# Autodesk Inventor assembly: DishBoard
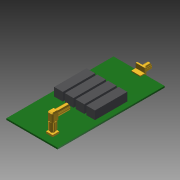
[picture p0: Inventor's stored thumbnail of the model, 180x180]
Saved by Autodesk Inventor 2014 (Build 180170000, 170)
## iProperties
Created: 2015-01-07
Part Number: DishBoard
Document SubType Name: Assembly
Designer: Owner
Author: Owner
## Documents named in this file (6)
- C:\Users\Owner\Documents\APC\FrontEnd\IAM\Dish\DishBoard.iam
- C:\Users\Owner\Documents\APC\FrontEnd\IAM\Dish\Dish_Board.ipt
- C:\Users\Owner\Documents\APC\FrontEnd\IAM\Common\SMA_Edge.ipt
- C:\Users\Owner\Documents\APC\FrontEnd\IAM\Common\SMA_Up.ipt
- C:\Users\Owner\Documents\APC\FrontEnd\IAM\Common\SMA_RightAngle.ipt
- C:\Users\Owner\Documents\APC\FrontEnd\IAM\Common\BPF.ipt
## Components (8 placed, 5 different names)
1. Dish_Board:1 — Mate:3, Mate:4, Flush:3, Mate:12, Mate:13, Mate:14, Mate:15, Mate:16, Flush:4, Flush:5, Flush:6, Flush:7, Flush:8, Flush:9, Flush:10, Flush:11
2. SMA_Edge:4 — Mate:3, Mate:4, Flush:3
3. SMA_Up:1 — Mate:10, Mate:11, Mate:12
4. SMA_RightAngle:1 — Mate:10, Mate:11
5. BPF:1 — Mate:13, Flush:7, Flush:11
6. BPF:2 — Mate:14, Flush:5, Flush:8
7. BPF:3 — Mate:15, Flush:4, Flush:10
8. BPF:4 — Mate:16, Flush:6, Flush:9
## Relationships (18: Mate 9, Flush 9)
- Mate:3: Dish_Board:1 ↔ SMA_Edge:4
- Mate:4: Dish_Board:1 ↔ SMA_Edge:4
- Flush:3 (-21.336 mm): Dish_Board:1 ↔ SMA_Edge:4
- Mate:10 (2 mm): SMA_Up:1 ↔ SMA_RightAngle:1
- Mate:11: SMA_Up:1 ↔ SMA_RightAngle:1
- Mate:12: Dish_Board:1 ↔ SMA_Up:1
- Mate:13: Dish_Board:1 ↔ BPF:1
- Mate:14: Dish_Board:1 ↔ BPF:2
- Mate:15: Dish_Board:1 ↔ BPF:3
- Mate:16: Dish_Board:1 ↔ BPF:4
- Flush:4 (34.2392 mm): Dish_Board:1 ↔ BPF:3
- Flush:5 (34.2392 mm): Dish_Board:1 ↔ BPF:2
- Flush:6 (34.2392 mm): Dish_Board:1 ↔ BPF:4
- Flush:7 (34.2392 mm): Dish_Board:1 ↔ BPF:1
- Flush:8 (5.6134 mm): Dish_Board:1 ↔ BPF:2
- Flush:9 (17.0434 mm): Dish_Board:1 ↔ BPF:4
- Flush:10 (28.4734 mm): Dish_Board:1 ↔ BPF:3
- Flush:11 (-39.9034 mm): Dish_Board:1 ↔ BPF:1
